# Autodesk Inventor assembly: Assembly-payload
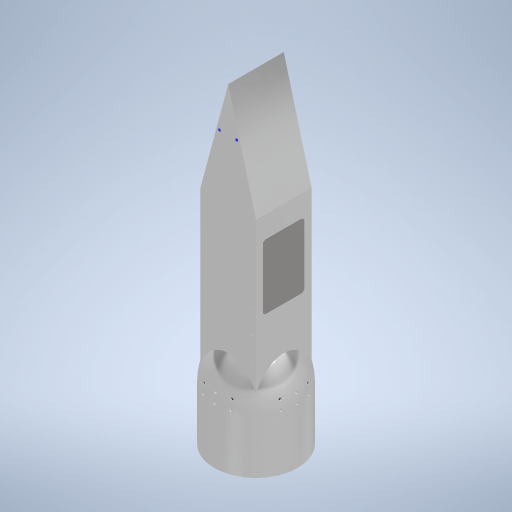
[picture p0: Inventor's stored thumbnail of the model, 512x512]
Saved by Autodesk Inventor 2023 (Build 270158000, 158)
## iProperties
Created: 2023-04-06
Part Number: Assembly-payload
Document SubType Name: Assembly
Designer: ASARe-DAQ-PC
Mass: 45573 g
Surface Area: 113214 cm^2
Volume: 33294.6 cm^3
Density: 1.36878 g/cm^3
Author: ASARe-DAQ-PC
## Documents named in this file (8)
- C:\Users\310611102\Documents\Inventor\SSR\avionics_2023ver\Payload\Assembly-payload.iam
- C:\Users\310611102\Documents\Inventor\SSR\avionics_2023ver\Payload\Assembly-payload-part1.iam
- C:\Users\310611102\Documents\Inventor\SSR\avionics_2023ver\Payload\Model Shell - access panel R.ipt
- C:\Users\310611102\Documents\Inventor\SSR\avionics_2023ver\Payload\Model Shell_part2.ipt
- C:\Users\310611102\Documents\Inventor\SSR\avionics_2023ver\Payload\Camera system.iam
- C:\Users\310611102\Documents\Inventor\SSR\avionics_2023ver\Payload\Screw M4 Hex Flat Head 14mm.ipt
- C:\Users\310611102\Documents\Inventor\SSR\avionics_2023ver\Payload\Screw M4 Hex 40mm.ipt
- C:\Users\310611102\Documents\Inventor\SSR\avionics_2023ver\Payload\Screw M3 Hex 8mm.ipt
## Components (65 placed, 7 different names)
1. Assembly-payload-part1:1 [sub-assembly] — Mate:3, Mate:4, Insert:7, Insert:20, Insert:21, Mate:5, Insert:118, Insert:119
2. Model Shell - access panel R:1 — Insert:20, Insert:21, Insert:24, Insert:25, Insert:26, Insert:27, Insert:28, Insert:29, Insert:30, Insert:31, Insert:32, Insert:33, Insert:34, Insert:35, Insert:36, Insert:37, Insert:38, Insert:39, Insert:40, Insert:41, Insert:42, Insert:43, Insert:44, Insert:45, Insert:46, Insert:47, Insert:48, Insert:49, Insert:50, Insert:51, Insert:52, Insert:53, Insert:54, Insert:55, Insert:56
3. Model Shell_part2:1 — Mate:3, Mate:4, Insert:7, Insert:90, Insert:91, Insert:92, Insert:93, Insert:94, Insert:95, Insert:96, Insert:97, Insert:98, Insert:99, Insert:100, Insert:101, Insert:102, Insert:103, Insert:104, Insert:105, Insert:106, Insert:107, Insert:108, Insert:109, Insert:110, Insert:111, Insert:112, Insert:113
4. Camera system:1 [sub-assembly] — Insert:114, Insert:115, Insert:116, Insert:117, Mate:5, Insert:118, Insert:119
5. Screw M4 Hex Flat Head 14mm:1 — Insert:43
6. Screw M4 Hex Flat Head 14mm:2 — Insert:42
7. Screw M4 Hex Flat Head 14mm:3 — Insert:44
8. Screw M4 Hex Flat Head 14mm:4 — Insert:45
9. Screw M4 Hex Flat Head 14mm:5 — Insert:46
10. Screw M4 Hex Flat Head 14mm:6 — Insert:47
11. Screw M4 Hex Flat Head 14mm:7 — Insert:48
12. Screw M4 Hex Flat Head 14mm:8 — Insert:49
13. Screw M4 Hex Flat Head 14mm:9 — Insert:50
14. Screw M4 Hex Flat Head 14mm:10 — Insert:51
15. Screw M4 Hex Flat Head 14mm:11 — Insert:52
16. Screw M4 Hex Flat Head 14mm:12 — Insert:53
17. Screw M4 Hex Flat Head 14mm:13 — Insert:54
18. Screw M4 Hex Flat Head 14mm:14 — Insert:55
19. Screw M4 Hex Flat Head 14mm:15 — Insert:24
20. Screw M4 Hex Flat Head 14mm:16 — Insert:25
21. Screw M4 Hex Flat Head 14mm:17 — Insert:26
22. Screw M4 Hex Flat Head 14mm:18 — Insert:27
23. Screw M4 Hex Flat Head 14mm:19 — Insert:28
24. Screw M4 Hex Flat Head 14mm:20 — Insert:29
25. Screw M4 Hex Flat Head 14mm:21 — Insert:30
26. Screw M4 Hex Flat Head 14mm:22 — Insert:31
27. Screw M4 Hex Flat Head 14mm:23 — Insert:32
28. Screw M4 Hex Flat Head 14mm:24 — Insert:33
29. Screw M4 Hex Flat Head 14mm:25 — Insert:34
30. Screw M4 Hex Flat Head 14mm:26 — Insert:35
31. Screw M4 Hex Flat Head 14mm:27 — Insert:36
32. Screw M4 Hex Flat Head 14mm:28 — Insert:37
33. Screw M4 Hex Flat Head 14mm:29 — Insert:38
34. Screw M4 Hex Flat Head 14mm:30 — Insert:41
35. Screw M4 Hex Flat Head 14mm:31 — Insert:40
36. Screw M4 Hex Flat Head 14mm:32 — Insert:39
37. Screw M4 Hex Flat Head 14mm:33 — Insert:56
38. Screw M4 Hex 40mm:1 — Insert:90
39. Screw M4 Hex 40mm:2 — Insert:92
40. Screw M4 Hex 40mm:3 — Insert:91
41. Screw M4 Hex 40mm:4 — Insert:93
42. Screw M4 Hex 40mm:5 — Insert:95
43. Screw M4 Hex 40mm:6 — Insert:94
44. Screw M4 Hex 40mm:7 — Insert:96
45. Screw M4 Hex 40mm:8 — Insert:97
46. Screw M4 Hex 40mm:9 — Insert:98
47. Screw M4 Hex 40mm:10 — Insert:99
48. Screw M4 Hex 40mm:11 — Insert:100
49. Screw M4 Hex 40mm:12 — Insert:101
50. Screw M4 Hex 40mm:13 — Insert:102
51. Screw M4 Hex 40mm:14 — Insert:103
52. Screw M4 Hex 40mm:15 — Insert:104
53. Screw M4 Hex 40mm:16 — Insert:105
54. Screw M4 Hex 40mm:17 — Insert:106
55. Screw M4 Hex 40mm:18 — Insert:107
56. Screw M4 Hex 40mm:19 — Insert:108
57. Screw M4 Hex 40mm:20 — Insert:109
58. Screw M4 Hex 40mm:21 — Insert:110
59. Screw M4 Hex 40mm:22 — Insert:111
60. Screw M4 Hex 40mm:23 — Insert:112
61. Screw M4 Hex 40mm:24 — Insert:113
62. Screw M3 Hex 8mm:1 — Insert:114
63. Screw M3 Hex 8mm:2 — Insert:115
64. Screw M3 Hex 8mm:3 — Insert:116
65. Screw M3 Hex 8mm:4 — Insert:117
## Relationships (69: Insert 66, Mate 3)
- Mate:3: Assembly-payload-part1:1 ↔ Model Shell_part2:1
- Mate:4: Assembly-payload-part1:1 ↔ Model Shell_part2:1
- Insert:7: Assembly-payload-part1:1 ↔ Model Shell_part2:1
- Insert:20: Assembly-payload-part1:1 ↔ Model Shell - access panel R:1
- Insert:21: Assembly-payload-part1:1 ↔ Model Shell - access panel R:1
- Insert:24: Model Shell - access panel R:1 ↔ Screw M4 Hex Flat Head 14mm:15
- Insert:25: Model Shell - access panel R:1 ↔ Screw M4 Hex Flat Head 14mm:16
- Insert:26: Model Shell - access panel R:1 ↔ Screw M4 Hex Flat Head 14mm:17
- Insert:27: Model Shell - access panel R:1 ↔ Screw M4 Hex Flat Head 14mm:18
- Insert:28: Model Shell - access panel R:1 ↔ Screw M4 Hex Flat Head 14mm:19
- Insert:29: Model Shell - access panel R:1 ↔ Screw M4 Hex Flat Head 14mm:20
- Insert:30: Model Shell - access panel R:1 ↔ Screw M4 Hex Flat Head 14mm:21
- Insert:31: Model Shell - access panel R:1 ↔ Screw M4 Hex Flat Head 14mm:22
- Insert:32: Model Shell - access panel R:1 ↔ Screw M4 Hex Flat Head 14mm:23
- Insert:33: Model Shell - access panel R:1 ↔ Screw M4 Hex Flat Head 14mm:24
- Insert:34: Model Shell - access panel R:1 ↔ Screw M4 Hex Flat Head 14mm:25
- Insert:35: Model Shell - access panel R:1 ↔ Screw M4 Hex Flat Head 14mm:26
- Insert:36: Model Shell - access panel R:1 ↔ Screw M4 Hex Flat Head 14mm:27
- Insert:37: Model Shell - access panel R:1 ↔ Screw M4 Hex Flat Head 14mm:28
- Insert:38: Model Shell - access panel R:1 ↔ Screw M4 Hex Flat Head 14mm:29
- Insert:39: Model Shell - access panel R:1 ↔ Screw M4 Hex Flat Head 14mm:32
- Insert:40: Model Shell - access panel R:1 ↔ Screw M4 Hex Flat Head 14mm:31
- Insert:41: Model Shell - access panel R:1 ↔ Screw M4 Hex Flat Head 14mm:30
- Insert:42: Model Shell - access panel R:1 ↔ Screw M4 Hex Flat Head 14mm:2
- Insert:43: Model Shell - access panel R:1 ↔ Screw M4 Hex Flat Head 14mm:1
- Insert:44: Model Shell - access panel R:1 ↔ Screw M4 Hex Flat Head 14mm:3
- Insert:45: Model Shell - access panel R:1 ↔ Screw M4 Hex Flat Head 14mm:4
- Insert:46: Model Shell - access panel R:1 ↔ Screw M4 Hex Flat Head 14mm:5
- Insert:47: Model Shell - access panel R:1 ↔ Screw M4 Hex Flat Head 14mm:6
- Insert:48: Model Shell - access panel R:1 ↔ Screw M4 Hex Flat Head 14mm:7
- Insert:49: Model Shell - access panel R:1 ↔ Screw M4 Hex Flat Head 14mm:8
- Insert:50: Model Shell - access panel R:1 ↔ Screw M4 Hex Flat Head 14mm:9
- Insert:51: Model Shell - access panel R:1 ↔ Screw M4 Hex Flat Head 14mm:10
- Insert:52: Model Shell - access panel R:1 ↔ Screw M4 Hex Flat Head 14mm:11
- Insert:53: Model Shell - access panel R:1 ↔ Screw M4 Hex Flat Head 14mm:12
- Insert:54: Model Shell - access panel R:1 ↔ Screw M4 Hex Flat Head 14mm:13
- Insert:55: Model Shell - access panel R:1 ↔ Screw M4 Hex Flat Head 14mm:14
- Insert:56: Model Shell - access panel R:1 ↔ Screw M4 Hex Flat Head 14mm:33
- Insert:90: Model Shell_part2:1 ↔ Screw M4 Hex 40mm:1
- Insert:91: Model Shell_part2:1 ↔ Screw M4 Hex 40mm:3
- Insert:92: Model Shell_part2:1 ↔ Screw M4 Hex 40mm:2
- Insert:93: Model Shell_part2:1 ↔ Screw M4 Hex 40mm:4
- Insert:94: Model Shell_part2:1 ↔ Screw M4 Hex 40mm:6
- Insert:95: Model Shell_part2:1 ↔ Screw M4 Hex 40mm:5
- Insert:96: Model Shell_part2:1 ↔ Screw M4 Hex 40mm:7
- Insert:97: Model Shell_part2:1 ↔ Screw M4 Hex 40mm:8
- Insert:98: Model Shell_part2:1 ↔ Screw M4 Hex 40mm:9
- Insert:99: Model Shell_part2:1 ↔ Screw M4 Hex 40mm:10
- Insert:100: Model Shell_part2:1 ↔ Screw M4 Hex 40mm:11
- Insert:101: Model Shell_part2:1 ↔ Screw M4 Hex 40mm:12
- Insert:102: Model Shell_part2:1 ↔ Screw M4 Hex 40mm:13
- Insert:103: Model Shell_part2:1 ↔ Screw M4 Hex 40mm:14
- Insert:104: Model Shell_part2:1 ↔ Screw M4 Hex 40mm:15
- Insert:105: Model Shell_part2:1 ↔ Screw M4 Hex 40mm:16
- Insert:106: Model Shell_part2:1 ↔ Screw M4 Hex 40mm:17
- Insert:107: Model Shell_part2:1 ↔ Screw M4 Hex 40mm:18
- Insert:108: Model Shell_part2:1 ↔ Screw M4 Hex 40mm:19
- Insert:109: Model Shell_part2:1 ↔ Screw M4 Hex 40mm:20
- Insert:110: Model Shell_part2:1 ↔ Screw M4 Hex 40mm:21
- Insert:111: Model Shell_part2:1 ↔ Screw M4 Hex 40mm:22
- Insert:112: Model Shell_part2:1 ↔ Screw M4 Hex 40mm:23
- Insert:113: Model Shell_part2:1 ↔ Screw M4 Hex 40mm:24
- Insert:114: Camera system:1 ↔ Screw M3 Hex 8mm:1
- Insert:115: Camera system:1 ↔ Screw M3 Hex 8mm:2
- Insert:116: Camera system:1 ↔ Screw M3 Hex 8mm:3
- Insert:117: Camera system:1 ↔ Screw M3 Hex 8mm:4
- Mate:5: Assembly-payload-part1:1 ↔ Camera system:1
- Insert:118: Assembly-payload-part1:1 ↔ Camera system:1
- Insert:119: Assembly-payload-part1:1 ↔ Camera system:1
